# Autodesk Inventor assembly: whole_setup
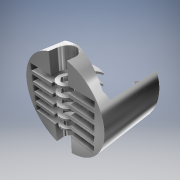
[picture p0: Inventor's stored thumbnail of the model, 180x180]
Saved by Autodesk Inventor 2016 (Build 200138000, 138)
## iProperties
Created: 2016-04-07
Part Number: whole_setup
Document SubType Name: Assembly
Designer: 3DPrinterUser
Author: 3DPrinterUser
## Documents named in this file (3)
- X:\Projekte Bastli\BarBot\BarBot\Conception\Mechanical\Ice_Dispenser\crusher\whole_setup.iam
- X:\Projekte Bastli\BarBot\BarBot\Conception\Mechanical\Ice_Dispenser\crusher\crusher_claw.ipt
- X:\Projekte Bastli\BarBot\BarBot\Conception\Mechanical\Ice_Dispenser\crusher\pipe_insertv2.ipt
## Components (6 placed, 2 different names)
1. crusher_claw:1 — Rotational:1
2. pipe_insertv2:1 — Rotational:1, Rotational:2, Rotational:3, Rotational:4, Rotational:5
3. crusher_claw:2 — Rotational:3
4. crusher_claw:3 — Rotational:2
5. crusher_claw:4 — Rotational:5
6. crusher_claw:5 — Rotational:4
## Relationships (5: RevoluteJoint 5)
- Rotational:1 [RevoluteJoint]: crusher_claw:1 ↔ pipe_insertv2:1
- Rotational:2 [RevoluteJoint]: pipe_insertv2:1 ↔ crusher_claw:3
- Rotational:3 [RevoluteJoint]: pipe_insertv2:1 ↔ crusher_claw:2
- Rotational:4 [RevoluteJoint]: pipe_insertv2:1 ↔ crusher_claw:5
- Rotational:5 [RevoluteJoint]: pipe_insertv2:1 ↔ crusher_claw:4
